# Autodesk Inventor assembly: Final_Assembly(KS-15)
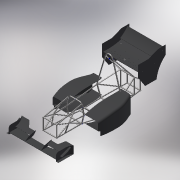
[picture p0: Inventor's stored thumbnail of the model, 180x180]
Saved by Autodesk Inventor 2018.2 (Build 222227000, 227)
## iProperties
Created: 2017-12-12
Part Number: Final_Assembly(KS-15)
Material: 一般
Document SubType Name: Assembly
Designer: kuwano
Author: kuwano
## Documents named in this file (6)
- D:\kuwano\Documents\Inventor\KITformula\AeroCAD2018\CAD\Inventor\Final_Assembly(KS-15).iam
- D:\kuwano\Documents\Inventor\KITformula\AeroCAD2018\CAD\Inventor\Assembly(KS-14.ver)\KS-15\frame2018.ipt
- D:\kuwano\Documents\Inventor\KITformula\AeroCAD2018\CAD\Inventor\製作用CAD\R-wing\R-wing.iam
- D:\kuwano\Documents\Inventor\KITformula\AeroCAD2018\CAD\Inventor\Aero Parts\F-wing\type7\F-wing.iam
- D:\kuwano\Documents\Inventor\KITformula\AeroCAD2018\CAD\Inventor\Aero Parts\Side Pontoon\type3(kuwano)\test.ipt
- D:\kuwano\Documents\Inventor\KITformula\AeroCAD2018\CAD\Inventor\Aero Parts\Side Pontoon\type3(kuwano)\test_MIR.ipt
## Components (5 placed, 5 different names)
1. frame2018:1 — メイト:1, メイト:2, メイト:3
2. R-wing:1 [sub-assembly] — フラッシュ:1, 角度:1
3. F-wing:1 [sub-assembly] — フラッシュ:2, 角度:2
4. test:1 — 角度:3, 角度:4, フラッシュ:3, メイト:4, メイト:5
5. test_MIR:1 — フラッシュ:3, メイト:4, メイト:5
## Relationships (12: Mate 5, Angle 4, Flush 3)
- メイト:1 [Mate]: frame2018:1
- メイト:2 [Mate]: frame2018:1
- メイト:3 [Mate]: frame2018:1
- フラッシュ:1 [Flush]: R-wing:1
- 角度:1 [Angle] (0 deg): R-wing:1
- フラッシュ:2 [Flush]: F-wing:1
- 角度:2 [Angle] (0 deg): F-wing:1
- 角度:3 [Angle] (0 deg): test:1
- 角度:4 [Angle] (0 deg): test:1
- フラッシュ:3 [Flush]: test:1 ↔ test_MIR:1
- メイト:4 [Mate]: test:1 ↔ test_MIR:1
- メイト:5 [Mate]: test:1 ↔ test_MIR:1
